# Autodesk Inventor assembly: 2016-01-23-RhinoRobotV02
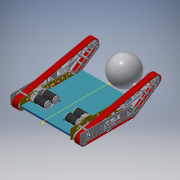
[picture p0: Inventor's stored thumbnail of the model, 180x180]
Saved by Autodesk Inventor 2016 SP1 (Build 200210100, 210)
## iProperties
Created: 2016-01-23
Part Number: 2016-01-23-RhinoRobotV02
Document SubType Name: Assembly
Designer: steele
Author: steele
## Documents named in this file (5)
- C:\snobotics\CAD-Development\robSteele\SnoBotics2016\2016-01-23-RhinoRobot\2016-01-23-RhinoRobotV02.iam
- C:\snobotics\CAD-Development\robSteele\SnoBotics2016\RhinoTrackDriveModule\am-3322+RhinoTrackDriveModule.iam
- C:\snobotics\CAD-Development\robSteele\SnoBotics2016\RhinoBottomFloorOptions\RhinoBottomFloorPlate02.ipt
- C:\snobotics\CAD-Development\robSteele\SnoBotics2016\DraftOfBoulder.ipt
- C:\snobotics\CAD-Development\robSteele\SnoBotics2016\RhinoTrackDriveModule\am-3322+RhinoTrackDriveModule_MIR5.iam
## Components (4 placed, 4 different names)
1. RhinoBottomFloorPlate02:1 — Mate:1, Flush:2, Flush:3, Mate:2
2. am-3322+RhinoTrackDriveModule:1 [sub-assembly] — Mate:1, Flush:2, Flush:3
3. DraftOfBoulder:1 — Mate:2, Mate:3
4. am-3322+RhinoTrackDriveModule_MIR5:1 [sub-assembly]
## Relationships (5: Mate 3, Flush 2)
- Mate:1 (3.175 mm): RhinoBottomFloorPlate02:1 ↔ am-3322+RhinoTrackDriveModule:1
- Flush:2: RhinoBottomFloorPlate02:1 ↔ am-3322+RhinoTrackDriveModule:1
- Flush:3 (48.26 mm): RhinoBottomFloorPlate02:1 ↔ am-3322+RhinoTrackDriveModule:1
- Mate:2: RhinoBottomFloorPlate02:1 ↔ DraftOfBoulder:1
- Mate:3 (-457.2 mm): DraftOfBoulder:1
## Named parameters: robotWidth = 660.4 mm, halfRobotWidth = 330.2 mm, maxPerimeter = 3048 mm, maxLength = 863.6 mm, widthOfTrack = 95.25 mm, boardWidth = 469.9 mm
